# Autodesk Inventor assembly: 外周ピンユニット
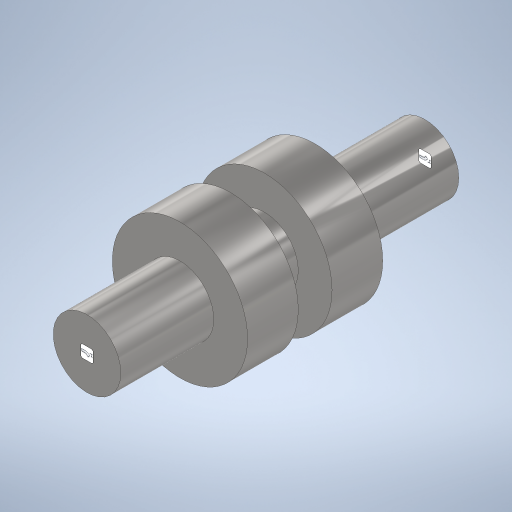
[picture p0: Inventor's stored thumbnail of the model, 512x512]
Saved by Autodesk Inventor 2024 (Build 280153000, 153)
## iProperties
Created: 2023-05-29
Part Number: 外周ピンユニット
Document SubType Name: Assembly
Designer: yuta2
Mass: 3.02791 g
Surface Area: 5.5292 cm^2
Volume: 0.380918 cm^3
Density: 7.94897 g/cm^3
Author: yuta2
## Documents named in this file (9)
- C:\Users\yuta2\Documents\Inventor\mokemoke2023\サイクロイド減速機_大型\外周ピンユニット.iam
- C:\Users\yuta2\Documents\Inventor\mokemoke2023\サイクロイド減速機_大型\外周ピン.ipt
- C:\Users\yuta2\Documents\Inventor\mokemoke2023\ベアリング\MF84ZZ.ipt
- C:\Users\yuta2\Documents\Inventor\mokemoke2023\サイクロイド減速機_大型\外周ピンユニット\AIP\FEA\ecmunh8n4.fins
- C:\Users\yuta2\Documents\Inventor\mokemoke2023\サイクロイド減速機_大型\外周ピンユニット\AIP\FEA\ecmunh8n4.fsat
- C:\Users\yuta2\Documents\Inventor\mokemoke2023\サイクロイド減速機_大型\外周ピンユニット\AIP\FEA\ecmunh8n4.ftes
- C:\Users\yuta2\Documents\Inventor\mokemoke2023\サイクロイド減速機_大型\外周ピンユニット\AIP\FEA\ecmunh8n4.fwiz
- C:\Users\yuta2\Documents\Inventor\mokemoke2023\サイクロイド減速機_大型\外周ピンユニット\AIP\FEA\ecmunh8n5.fmsh
- C:\Users\yuta2\Documents\Inventor\mokemoke2023\サイクロイド減速機_大型\外周ピンユニット\AIP\FEA\ecmunh8n6.fres
## Components (3 placed, 2 different names)
1. 外周ピン:1 — 回転:1
2. MF84ZZ:1 — 回転:1, 回転:2
3. MF84ZZ:2 — 回転:2
## Relationships (2: RevoluteJoint 2)
- 回転:1 [RevoluteJoint] (-6.5 mm): 外周ピン:1 ↔ MF84ZZ:1
- 回転:2 [RevoluteJoint] (2 mm): MF84ZZ:1 ↔ MF84ZZ:2
## Named parameters: sa_0 = 150000
note: some values were not read from the file. Shown as the stored number, unit unknown: "sa_0".
